# Autodesk Inventor assembly: Arm
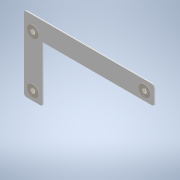
[picture p0: Inventor's stored thumbnail of the model, 180x180]
Saved by Autodesk Inventor 2020 (Build 240168000, 168)
## iProperties
Created: 2020-01-26
Part Number: Arm
Document SubType Name: Assembly
Designer: autum
Author: autum
## Documents named in this file (3)
- C:\Users\autum\Google Drive\Iron Riders 4180 (Roosevelt Robotics)\2019-2020\Build_Design\Robot 2020 (new)\Intake 2.0\Arm.iam
- C:\Users\autum\Google Drive\Iron Riders 4180 (Roosevelt Robotics)\2019-2020\Build_Design\Robot 2020 (new)\Intake 2.0\Arm.ipt
- C:\Users\autum\Google Drive\Iron Riders 4180 (Roosevelt Robotics)\2019-2020\Build_Design\Robot 2020 (new)\Intake 2.0\Hex Bearing.ipt
## Components (4 placed, 2 different names)
1. Arm:1 — Insert:1, Insert:2, Insert:3
2. Hex Bearing:1 — Insert:1
3. Hex Bearing:2 — Insert:2
4. Hex Bearing:3 — Insert:3
## Relationships (3: Insert 3)
- Insert:1: Arm:1 ↔ Hex Bearing:1
- Insert:2: Arm:1 ↔ Hex Bearing:2
- Insert:3: Arm:1 ↔ Hex Bearing:3
